# Autodesk Inventor assembly: VF1 TABLE + FLEX_KURT D688
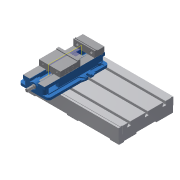
[picture p0: Inventor's stored thumbnail of the model, 180x180]
Saved by Autodesk Inventor 2021.4 (Build 254397000, 397)
## iProperties
Created: 2022-03-02
Part Number: VF1 TABLE + FLEX_KURT D688
Document SubType Name: Assembly
Designer: rodar
Author: rodar
## Documents named in this file (3)
- C:\Users\rodar\OneDrive\Desktop\INVENTOR\UVG\EQUIPO TALLER\VF1 TABLE + FLEX_KURT D688.iam
- C:\Users\rodar\OneDrive\Desktop\INVENTOR\UVG\EQUIPO TALLER\HAAS\VF -1\VF-1_Table.ipt
- C:\Users\rodar\OneDrive\Desktop\INVENTOR\UVG\EQUIPO TALLER\WORK HOLDING\KURT\FLEX_KURT D688.iam
## Components (2 placed, 2 different names)
1. VF-1_Table:1 — Mate:1, Flush:3, Flush:4
2. FLEX_KURT D688:1 [sub-assembly] — Mate:1, Flush:3, Flush:4
## Relationships (3: Flush 2, Mate 1)
- Mate:1: VF-1_Table:1 ↔ FLEX_KURT D688:1
- Flush:3 (-175 mm): VF-1_Table:1 ↔ FLEX_KURT D688:1
- Flush:4: VF-1_Table:1 ↔ FLEX_KURT D688:1
